# Autodesk Inventor assembly: Case_Principal_3
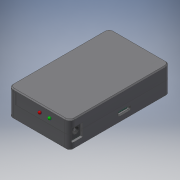
[picture p0: Inventor's stored thumbnail of the model, 180x180]
Saved by Autodesk Inventor 2019 (Build 230136000, 136)
## iProperties
Created: 2018-11-27
Part Number: Case_Principal_3
Document SubType Name: Assembly
Designer: DIEGO 01
Author: DIEGO 01
## Documents named in this file (7)
- D:\Hector\CAD_thesis\Case_Principal_3.iam
- D:\Hector\CAD_thesis\Case\Case_3_inferior.ipt
- D:\Hector\CAD_thesis\PCB\tesis_schematic.iam
- D:\Hector\CAD_thesis\Case\Case_3_superior.ipt
- D:\Hector\CAD_thesis\intento1.ipt
- D:\Hector\CAD_thesis\LED\LED_3MM_ROJO.ipt
- D:\Hector\CAD_thesis\LED\LED_3MM_VERDE.ipt
## Components (6 placed, 6 different names)
1. Case_3_inferior:1 — Nivelación:1, Nivelación:2, Nivelación:3, Coincidencia:1, Coincidencia:2, Coincidencia:3, Coincidencia:4, Nivelación:4, Nivelación:5, Nivelación:6, Coincidencia:5, Coincidencia:6
2. tesis_schematic:1 [sub-assembly] — Coincidencia:1, Coincidencia:2, Coincidencia:3
3. Case_3_superior:1 — Coincidencia:4, Nivelación:4, Nivelación:5, Coincidencia:7, Coincidencia:8, Coincidencia:9, Nivelación:8
4. intento1:1 — Nivelación:6, Coincidencia:5, Coincidencia:6
5. LED_3MM_ROJO:1 — Coincidencia:8, Nivelación:7, Coincidencia:9, Nivelación:9
6. LED_3MM_VERDE:1 — Coincidencia:7, Nivelación:7, Nivelación:8, Nivelación:9
## Relationships (18: Flush 9, Mate 9)
- Nivelación:1 [Flush]: Case_3_inferior:1
- Nivelación:2 [Flush]: Case_3_inferior:1
- Nivelación:3 [Flush]: Case_3_inferior:1
- Coincidencia:1 [Mate]: Case_3_inferior:1 ↔ tesis_schematic:1
- Coincidencia:2 [Mate] (0.5 mm): Case_3_inferior:1 ↔ tesis_schematic:1
- Coincidencia:3 [Mate] (0.5 mm): Case_3_inferior:1 ↔ tesis_schematic:1
- Coincidencia:4 [Mate]: Case_3_inferior:1 ↔ Case_3_superior:1
- Nivelación:4 [Flush]: Case_3_inferior:1 ↔ Case_3_superior:1
- Nivelación:5 [Flush]: Case_3_inferior:1 ↔ Case_3_superior:1
- Nivelación:6 [Flush] (-0.3 mm): Case_3_inferior:1 ↔ intento1:1
- Coincidencia:5 [Mate] (-9 mm): Case_3_inferior:1 ↔ intento1:1
- Coincidencia:6 [Mate] (-15.75 mm): Case_3_inferior:1 ↔ intento1:1
- Coincidencia:7 [Mate]: Case_3_superior:1 ↔ LED_3MM_VERDE:1
- Coincidencia:8 [Mate]: Case_3_superior:1 ↔ LED_3MM_ROJO:1
- Nivelación:7 [Flush]: LED_3MM_ROJO:1 ↔ LED_3MM_VERDE:1
- Coincidencia:9 [Mate] (-6.8 mm): Case_3_superior:1 ↔ LED_3MM_ROJO:1
- Nivelación:8 [Flush] (20 mm): Case_3_superior:1 ↔ LED_3MM_VERDE:1
- Nivelación:9 [Flush] (-10 mm): LED_3MM_ROJO:1 ↔ LED_3MM_VERDE:1
